# Autodesk Inventor assembly: Motor
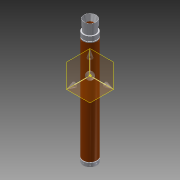
[picture p0: Inventor's stored thumbnail of the model, 180x180]
Saved by Autodesk Inventor 2015 (Build 190159000, 159)
## iProperties
Created: 2016-01-09
Part Number: Motor
Document SubType Name: Assembly
Designer: Jared
Mass: 8113.68 g
Surface Area: 13872.5 cm^2
Volume: 4793.75 cm^3
Density: 1.69255 g/cm^3
Author: Jared
## Documents named in this file (5)
- D:\Google Drive\TRC Members\3. IPT (Integrated Product Teams)\Propulsion\2015-2016 Year\6 in Motor\CAD\Flight Motor\Version 2\Motor.iam
- D:\Google Drive\TRC Members\3. IPT (Integrated Product Teams)\Propulsion\2015-2016 Year\6 in Motor\CAD\Flight Motor\Version 2\Forward Closure.ipt
- D:\Google Drive\TRC Members\3. IPT (Integrated Product Teams)\Propulsion\2015-2016 Year\6 in Motor\CAD\Flight Motor\Version 2\Liner.ipt
- D:\Google Drive\TRC Members\3. IPT (Integrated Product Teams)\Propulsion\2015-2016 Year\6 in Motor\CAD\Flight Motor\Version 2\Upper Thermal Barrier.ipt
- D:\Google Drive\TRC Members\3. IPT (Integrated Product Teams)\Propulsion\2015-2016 Year\6 in Motor\CAD\Flight Motor\Version 2\Nozzle.iam
## Components (4 placed, 4 different names)
1. Forward Closure:1 — Mate:3, Mate:4, Mate:7
2. Liner:1 — Mate:1, Mate:2, Mate:4, Mate:5, Mate:6, Mate:8, Mate:9
3. Upper Thermal Barrier:1 — Mate:1, Mate:2, Mate:3
4. Nozzle:1 [sub-assembly] — Mate:5, Mate:6, Mate:9
## Relationships (9: Mate 9)
- Mate:1: Liner:1 ↔ Upper Thermal Barrier:1
- Mate:2: Liner:1 ↔ Upper Thermal Barrier:1
- Mate:3: Forward Closure:1 ↔ Upper Thermal Barrier:1
- Mate:4: Forward Closure:1 ↔ Liner:1
- Mate:5: Liner:1 ↔ Nozzle:1
- Mate:6: Liner:1 ↔ Nozzle:1
- Mate:7: Forward Closure:1
- Mate:8: Liner:1
- Mate:9: Liner:1 ↔ Nozzle:1
